# Autodesk Inventor assembly: Slide Assembly V2
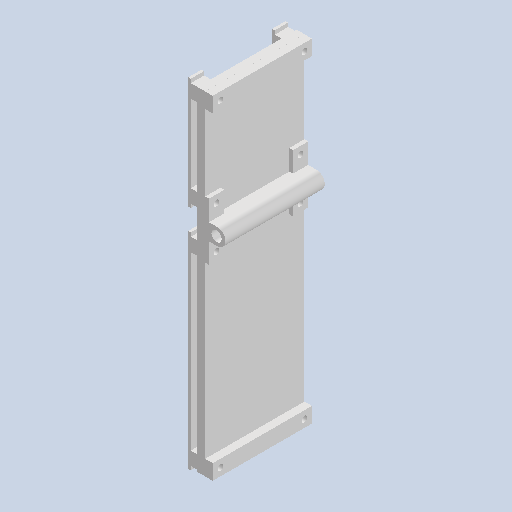
[picture p0: Inventor's stored thumbnail of the model, 512x512]
Saved by Autodesk Inventor 2025 (Build 290162000, 162)
## iProperties
Created: 2024-11-04
Part Number: Slide Assembly V2
Document SubType Name: Assembly
Designer: liaco
Author: liaco
## Documents named in this file (6)
- C:\Users\liaco\OneDrive\Documents\Graphics Labs\1P13 CAD Models\Design 2\Slide Assembly V2.iam
- C:\Users\liaco\OneDrive\Documents\Graphics Labs\1P13 CAD Models\Design 2\Tilt Slide V2.ipt
- C:\Users\liaco\OneDrive\Documents\Graphics Labs\1P13 CAD Models\Design 2\Axle Hold.ipt
- C:\Users\liaco\OneDrive\Documents\Graphics Labs\1P13 CAD Models\Design 2\Slide Block Short.ipt
- C:\Users\liaco\OneDrive\Documents\Graphics Labs\1P13 CAD Models\Design 2\Weight.ipt
- C:\Users\liaco\OneDrive\Documents\Graphics Labs\1P13 CAD Models\Design 2\Slide Block Long.ipt
## Components (8 placed, 5 different names)
1. Tilt Slide V2:1 — Mate:9, Mate:10, Mate:11, Mate:12, Mate:13, Mate:14, Mate:16, Mate:18, Mate:19, Mate:20, Mate:21, Mate:22, Mate:23, Mate:24, Mate:25, Mate:26, Mate:28
2. Axle Hold:1 — Mate:9, Mate:10, Mate:11, Mate:15, Mate:17, Mate:29
3. Slide Block Short:1 — Mate:13, Mate:14, Mate:15
4. Slide Block Short:2 — Mate:12, Mate:16, Mate:17
5. Weight:1 — Mate:19, Mate:20, Mate:22
6. Weight:2 — Mate:18, Mate:21, Mate:23, Mate:27
7. Slide Block Long:1 — Mate:24, Mate:26, Mate:27
8. Slide Block Long:2 — Mate:25, Mate:28, Mate:29
## Relationships (21: Mate 21)
- Mate:9: Tilt Slide V2:1 ↔ Axle Hold:1
- Mate:10: Tilt Slide V2:1 ↔ Axle Hold:1
- Mate:11: Tilt Slide V2:1 ↔ Axle Hold:1
- Mate:12: Tilt Slide V2:1 ↔ Slide Block Short:2
- Mate:13: Tilt Slide V2:1 ↔ Slide Block Short:1
- Mate:14: Tilt Slide V2:1 ↔ Slide Block Short:1
- Mate:15: Axle Hold:1 ↔ Slide Block Short:1
- Mate:16: Tilt Slide V2:1 ↔ Slide Block Short:2
- Mate:17: Axle Hold:1 ↔ Slide Block Short:2
- Mate:18: Tilt Slide V2:1 ↔ Weight:2
- Mate:19: Tilt Slide V2:1 ↔ Weight:1
- Mate:20: Tilt Slide V2:1 ↔ Weight:1
- Mate:21: Tilt Slide V2:1 ↔ Weight:2
- Mate:22: Tilt Slide V2:1 ↔ Weight:1
- Mate:23: Tilt Slide V2:1 ↔ Weight:2
- Mate:24: Tilt Slide V2:1 ↔ Slide Block Long:1
- Mate:25: Tilt Slide V2:1 ↔ Slide Block Long:2
- Mate:26: Tilt Slide V2:1 ↔ Slide Block Long:1
- Mate:27: Weight:2 ↔ Slide Block Long:1
- Mate:28: Tilt Slide V2:1 ↔ Slide Block Long:2
- Mate:29: Axle Hold:1 ↔ Slide Block Long:2
